# Autodesk Inventor assembly: sheetB
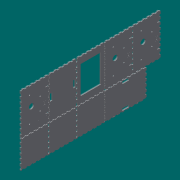
[picture p0: Inventor's stored thumbnail of the model, 180x180]
Saved by Autodesk Inventor 2016 SP2 (Build 200236200, 236)
## iProperties
Created: 2016-09-27
Part Number: sheetB
Document SubType Name: Assembly
Designer: sawaiz
Author: sawaiz
## Documents named in this file (8)
- C:\Users\sawaiz\OneDrive\projects\splitFlapDisplay\sheetB.iam
- C:\Users\sawaiz\oneDrive\projects\splitFlapDisplay\frame\leftSide.ipt
- C:\Users\sawaiz\oneDrive\projects\splitFlapDisplay\frame\back.ipt
- C:\Users\sawaiz\oneDrive\projects\splitFlapDisplay\frame\front.ipt
- C:\Users\sawaiz\oneDrive\projects\splitFlapDisplay\frame\topBottomPanel.ipt
- C:\Users\sawaiz\oneDrive\projects\splitFlapDisplay\frame\rightSide.ipt
- C:\Users\sawaiz\oneDrive\projects\splitFlapDisplay\sheetB.ipt
- C:\Users\sawaiz\oneDrive\projects\splitFlapDisplay\parameters.xlsx
## Components (10 placed, 6 different names)
1. leftSide:1 — Flush:1, Flush:2, Flush:3, Flush:4, Flush:5, Flush:10, Mate:3, Flush:13, Mate:5, Flush:22
2. back:1 — Flush:3, Flush:5, Flush:6, Flush:9, Flush:10, Mate:2, Mate:3, Flush:23
3. front:1 — Flush:2, Flush:6, Flush:7, Mate:1, Flush:8, Flush:9, Mate:2, Flush:15, Flush:24
4. topBottomPanel:1 — Flush:4, Flush:13, Mate:5, Flush:14, Flush:16, Mate:6, Flush:28
5. rightSide:1 — Flush:1, Flush:7, Mate:1, Flush:8, Mate:10, Flush:19, Flush:20, Mate:11, Flush:25
6. topBottomPanel:2 — Flush:14, Flush:16, Flush:17, Mate:6, Mate:7, Flush:26
7. topBottomPanel:3 — Flush:15, Flush:17, Mate:7, Flush:21, Mate:12, Flush:27
8. rightSide:2 — Mate:10, Flush:19, Flush:20, Flush:30
9. back:2 — Flush:21, Mate:11, Mate:12, Flush:29
10. sheetB:1 — Flush:22, Flush:23, Flush:24, Flush:25, Flush:26, Flush:27, Flush:28, Flush:29, Flush:30
## Relationships (36: Flush 27, Mate 9)
- Flush:1: leftSide:1 ↔ rightSide:1
- Flush:2: leftSide:1 ↔ front:1
- Flush:3: leftSide:1 ↔ back:1
- Flush:4: leftSide:1 ↔ topBottomPanel:1
- Flush:5: leftSide:1 ↔ back:1
- Flush:6: back:1 ↔ front:1
- Flush:7: front:1 ↔ rightSide:1
- Mate:1 (0.36 mm): front:1 ↔ rightSide:1
- Flush:8: front:1 ↔ rightSide:1
- Flush:9: back:1 ↔ front:1
- Flush:10: leftSide:1 ↔ back:1
- Mate:2 (0.36 mm): back:1 ↔ front:1
- Mate:3 (0.36 mm): leftSide:1 ↔ back:1
- Flush:13: leftSide:1 ↔ topBottomPanel:1
- Mate:5 (0.36 mm): leftSide:1 ↔ topBottomPanel:1
- Flush:14: topBottomPanel:1 ↔ topBottomPanel:2
- Flush:15: front:1 ↔ topBottomPanel:3
- Flush:16: topBottomPanel:1 ↔ topBottomPanel:2
- Flush:17: topBottomPanel:2 ↔ topBottomPanel:3
- Mate:6 (0.36 mm): topBottomPanel:1 ↔ topBottomPanel:2
- Mate:7 (0.36 mm): topBottomPanel:2 ↔ topBottomPanel:3
- Mate:10 (0.36 mm): rightSide:1 ↔ rightSide:2
- Flush:19: rightSide:1 ↔ rightSide:2
- Flush:20: rightSide:1 ↔ rightSide:2
- Flush:21: topBottomPanel:3 ↔ back:2
- Mate:11 (0.36 mm): rightSide:1 ↔ back:2
- Mate:12 (0.36 mm): topBottomPanel:3 ↔ back:2
- Flush:22: leftSide:1 ↔ sheetB:1
- Flush:23: back:1 ↔ sheetB:1
- Flush:24: front:1 ↔ sheetB:1
- Flush:25: rightSide:1 ↔ sheetB:1
- Flush:26: topBottomPanel:2 ↔ sheetB:1
- Flush:27: topBottomPanel:3 ↔ sheetB:1
- Flush:28: topBottomPanel:1 ↔ sheetB:1
- Flush:29: back:2 ↔ sheetB:1
- Flush:30: rightSide:2 ↔ sheetB:1
## Named parameters: height = 180 mm, width = 120 mm, depth = 120 mm, materialThickness = 3.175 mm, laserKerf = 0.12 mm, spoolDiameter = 90 mm, cardPinDiameter = 3 mm, cardNumber = 40, centeralShaftDiameter = 8 mm, cardWidth = 85.6 mm, cardHeight = 53.98 mm, cardThickness = 0.76 mm, cardFillet = 2.88 mm, cardCutoutHeight = 20 mm, cardClearence = 0.5 mm, spoolHubDiameter = 20 mm, bearingOd = 22 mm, bearingWidth = 8 mm, axleHeight = 95 mm, nutTrapClearence = 2 mm, nutTrapwidth = 5.5 mm, nutTrapDepth = 2.5 mm, beltLength = 240 mm, magnetDiameter = 6 mm, magnetLength = 3 mm, magnetProtusion = 0.25 mm, notchWidth = 10 mm, spoolThickness = 5.588 mm
